# Autodesk Inventor assembly: Hook Encoder Assembly
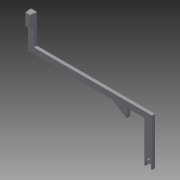
[picture p0: Inventor's stored thumbnail of the model, 180x180]
Saved by Autodesk Inventor 2013 (Build 170138000, 138)
## iProperties
Created: 2013-03-16
Part Number: Hook Encoder Assembly
Document SubType Name: Assembly
Designer: Arpan
Author: Arpan
## Documents named in this file (3)
- C:\Users\Arpan\Documents\GitHub\frc2013CAD\Midwest Climber\Hook Encoder Assembly.iam
- C:\Users\Arpan\Documents\GitHub\frc2013CAD\Midwest Climber\Limit Switch.ipt
- C:\Users\Arpan\Documents\GitHub\frc2013CAD\Midwest Climber\Left Climber Hook_v2.ipt
## Components (2 placed, 2 different names)
1. Limit Switch:1 — Flush:1, Flush:2, Mate:1
2. Left Climber Hook_v2:1 — Flush:1, Flush:2, Mate:1
## Relationships (3: Flush 2, Mate 1)
- Flush:1: Limit Switch:1 ↔ Left Climber Hook_v2:1
- Flush:2 (1.5875 mm): Limit Switch:1 ↔ Left Climber Hook_v2:1
- Mate:1: Limit Switch:1 ↔ Left Climber Hook_v2:1
